# Autodesk Inventor assembly: robot arm
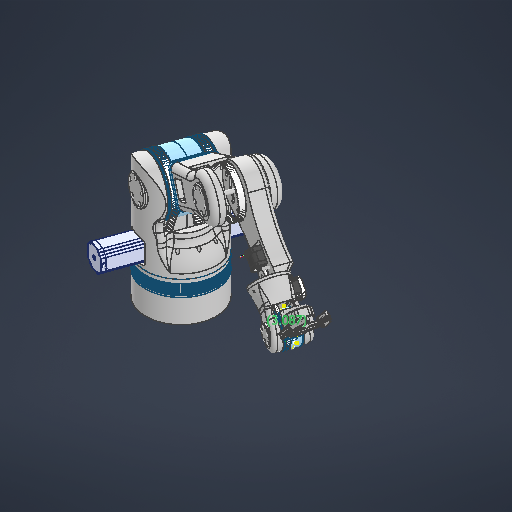
[picture p0: Inventor's stored thumbnail of the model, 512x512]
Saved by Autodesk Inventor 2026 (Build 300175000, 175)
## iProperties
Created: 2026-04-20
Part Number: robot arm
Document SubType Name: Assembly
Designer: oleg2
Author: oleg2
## Documents named in this file (35)
- E:\robot arm.iam
- E:\fasteners\m5 lock nut.ipt
- E:\fasteners\m5 washer.ipt
- E:\fasteners\m5 30mm screw.ipt
- E:\bottom piece.ipt
- E:\118t pulley part 2.ipt
- E:\bearing\outerbearingwheel.ipt
- E:\bearing\innerbearingwheel.ipt
- E:\middle piece.ipt
- E:\stepper motor.ipt
- E:\fasteners\m4 30mm screw.ipt
- E:\fasteners\m4 16mm flat head screw.ipt
- E:\fasteners\m5 hex nut.ipt
- E:\fasteners\m5 15mm screw.ipt
- E:\90t 1in pulley.ipt
- E:\rod.ipt
- E:\rodbearing.ipt
- E:\bearingplate.ipt
- E:\stepper motor 2.ipt
- E:\bearing 2.ipt
- E:\bearingplate 2.ipt
- E:\10mm rod.ipt
- E:\BELT LARGE.ipt
- E:\75t pulley (1).ipt
- E:\75t pulley right.ipt
- E:\final joint.ipt
- E:\3in 10mm rod.ipt
- E:\stepper 3.ipt
- E:\50t pulley.ipt
- E:\50t pulley right piece.ipt
- E:\bearing plate final.ipt
- E:\arm 2 fixed.ipt
- E:\epic claw.iam
- E:\107t belt.ipt
- E:\61t belt.ipt
## Components (115 placed, 34 different names)
1. m5 lock nut:1 — Mate:32, Mate:38
2. m5 washer:1 — Mate:20, Mate:24, Mate:39
3. m5 30mm screw:1 — Mate:10, Mate:12, Mate:26, Mate:33
4. bottom piece:1 — Mate:1, Mate:2, Mate:3, Mate:4, Mate:237
5. 118t pulley part 2:1 — Mate:1, Mate:6, Mate:18, Mate:19, Mate:20, Mate:21, Mate:22, Mate:23, Mate:24, Mate:25, Mate:40, Mate:41, Mate:42
6. outerbearingwheel:1 — Mate:2, Mate:3, Mate:4, Mate:5, Flush:1, Mate:61, Mate:62, Mate:63, Mate:64, Mate:65, Mate:66, Mate:67, Mate:68
7. innerbearingwheel:1 — Mate:5, Flush:1, Mate:6, Mate:7, Mate:8, Mate:9, Mate:10, Mate:15, Mate:16, Mate:17, Mate:25, Mate:27
8. m5 30mm screw:2 — Mate:7, Mate:11, Mate:29, Mate:32
9. m5 30mm screw:3 — Mate:8, Mate:14, Mate:30, Mate:31, Mate:35
10. m5 30mm screw:4 — Mate:9, Mate:13, Mate:28, Mate:34
11. m5 washer:2 — Mate:19, Mate:23, Mate:38
12. m5 washer:3 — Mate:18, Mate:31, Mate:36
13. m5 washer:4 — Mate:13, Mate:27, Mate:28
14. m5 washer:5 — Mate:12, Mate:16, Mate:26
15. m5 washer:6 — Mate:11, Mate:15, Mate:29
16. m5 washer:7 — Mate:14, Mate:17, Mate:30
17. m5 washer:8 — Mate:21, Mate:22, Mate:37
18. m5 lock nut:2 — Mate:33, Mate:39
19. m5 lock nut:3 — Mate:34, Mate:37
20. m5 lock nut:4 — Mate:35, Mate:36
21. middle piece:1 — Mate:40, Mate:41, Mate:42, Mate:43, Mate:44, Mate:45, Mate:46, Mate:47, Mate:48, Mate:49, Mate:50, Mate:51, Mate:52, Mate:53, Mate:54, Mate:55, Mate:56, Mate:57, Mate:58, Mate:59, Mate:60, Mate:69, Angle:1, Mate:70, Mate:71, Angle:2, Mate:72, Mate:73, Angle:3, Mate:74, Mate:75, Angle:4, Mate:76, Mate:77, Angle:5, Mate:78, Mate:79, Angle:6, Mate:80, Mate:81, Angle:7, Mate:82, Mate:83, Angle:8, Mate:84, Mate:89, Mate:104, Flush:3, Mate:130, Mate:131, Mate:203, Mate:205, Mate:206, Mate:238, Mate:239
22. stepper motor:1 — Mate:43, Mate:44, Mate:45, Mate:85, Mate:86, Mate:88, Mate:90, Mate:91, Mate:92, Mate:211
23. stepper motor:2 — Mate:46, Mate:47, Mate:48, Mate:93, Mate:94, Mate:95, Mate:96, Mate:97, Mate:98, Mate:99, Mate:100, Mate:208
24. m4 30mm screw:1 — Mate:49, Mate:50
25. m4 30mm screw:2 — Mate:51, Mate:52
26. m4 30mm screw:3 — Mate:53, Mate:54
27. m4 30mm screw:4 — Mate:55, Mate:56
28. m4 30mm screw:5 — Mate:57, Mate:58
29. m4 30mm screw:6 — Mate:59, Mate:60
30. m4 16mm flat head screw:1 — Mate:63, Mate:64
31. m4 16mm flat head screw:2 — Mate:61, Mate:62
32. m4 16mm flat head screw:3 — Mate:67, Mate:68
33. m4 16mm flat head screw:4 — Mate:65, Mate:66
34. m5 hex nut:1 — Mate:69, Angle:1, Mate:70
35. m5 hex nut:2 — Mate:71, Angle:2, Mate:72, Mate:87
36. m5 hex nut:3 — Mate:83, Angle:8, Mate:84
37. m5 hex nut:4 — Mate:81, Angle:7, Mate:82
38. m5 hex nut:5 — Mate:73, Angle:3, Mate:74
39. m5 hex nut:6 — Mate:75, Angle:4, Mate:76
40. m5 hex nut:7 — Mate:77, Angle:5, Mate:78
41. m5 hex nut:8 — Mate:79, Angle:6, Mate:80
42. m5 15mm screw:1 — Mate:91, Mate:92
43. m5 15mm screw:2 — Mate:87, Mate:88
44. m5 15mm screw:3 — Mate:93, Mate:94
45. m5 15mm screw:4 — Mate:89, Mate:90
46. m5 15mm screw:5 — Mate:97, Mate:98
47. m5 15mm screw:6 — Mate:95, Mate:96
48. m5 15mm screw:7 — Mate:99, Mate:100
49. m5 15mm screw:8 — Mate:85, Mate:86
50. 90t 1in pulley:1 — Mate:103, Mate:107, Mate:108, Mate:127, Mate:209, Mate:292
51. 90t 1in pulley:2 — Mate:103, Mate:104, Mate:107, Mate:119, Mate:120, Mate:121, Mate:122, Mate:123, Mate:124, Mate:125, Mate:126, Mate:127, Mate:212, Mate:291, Mate:293
52. rod:1 — Mate:108, Flush:3, Mate:109, Mate:111, Mate:113, Mate:118, Mate:203, Mate:207, Mate:210
53. rodbearing:1 — Mate:109, Mate:206
54. rodbearing:2 — Mate:111, Mate:205
55. bearingplate:1 — Mate:113, Mate:130, Mate:142, Mate:143, Mate:144, Mate:145, Mate:146, Mate:147, Mate:148, Mate:149, Mate:150, Mate:151
56. bearingplate:2 — Mate:118, Mate:131, Mate:132, Mate:133, Mate:134, Mate:135, Mate:136, Mate:137, Mate:138, Mate:139, Mate:140, Mate:141
57. m4 30mm screw:7 — Mate:119, Mate:120
58. m4 30mm screw:8 — Mate:121, Mate:122
59. m4 30mm screw:9 — Mate:123, Mate:124
60. m4 30mm screw:10 — Mate:125, Mate:126
61. m4 16mm flat head screw:5 — Mate:132, Mate:133, Mate:238
62. m4 16mm flat head screw:6 — Mate:134, Mate:135
63. m4 16mm flat head screw:7 — Mate:136, Mate:137
64. m4 16mm flat head screw:8 — Mate:150, Mate:151
65. m4 16mm flat head screw:9 — Mate:140, Mate:141
66. m4 16mm flat head screw:10 — Mate:138, Mate:139
67. m4 16mm flat head screw:12 — Mate:148, Mate:149
68. m4 16mm flat head screw:13 — Mate:142, Mate:143
69. m4 16mm flat head screw:14 — Mate:144, Mate:145
70. m4 16mm flat head screw:15 — Mate:146, Mate:147, Mate:239
71. stepper motor 2:1 — Mate:294, Mate:295, Mate:296, Mate:318
72. bearing 2:2 — Mate:175, Mate:290, Mate:299
73. bearingplate 2:1 — Mate:183, Mate:184, Mate:185, Mate:186, Mate:187, Mate:188, Mate:189, Mate:190, Mate:191, Mate:192, Mate:306
74. bearingplate 2:2 — Mate:175, Mate:193, Mate:194, Mate:195, Mate:196, Mate:197, Mate:198, Mate:199, Mate:200, Mate:201, Mate:202, Mate:204, Mate:300
75. 10mm rod:1 — Mate:290, Mate:302, Mate:311, Flush:5, Mate:317
76. m4 16mm flat head screw:16 — Mate:185, Mate:186
77. m4 16mm flat head screw:17 — Mate:187, Mate:188, Mate:304
78. m4 16mm flat head screw:18 — Mate:189, Mate:190, Mate:305
79. m4 16mm flat head screw:19 — Mate:195, Mate:196
80. m4 16mm flat head screw:20 — Mate:197, Mate:198
81. m4 16mm flat head screw:21 — Mate:201, Mate:202, Mate:204
82. m4 16mm flat head screw:22 — Mate:199, Mate:200
83. m4 16mm flat head screw:23 — Mate:193, Mate:194
84. m4 16mm flat head screw:24 — Mate:191, Mate:192
85. m4 16mm flat head screw:25 — Mate:183, Mate:184
86. BELT LARGE:1 — Mate:207, Mate:208, Mate:209
87. BELT LARGE:2 — Mate:210, Mate:211, Mate:212
88. 75t pulley (1):2 — Mate:236, Mate:250, Mate:308, Mate:309, Mate:320, Mate:322, Mate:323
89. stepper motor 2:2 — Mate:236, Mate:320, Mate:321
90. 75t pulley right:2 — Mate:307, Mate:308, Mate:309, Mate:310, Mate:313, Mate:321
91. final joint:1 — Mate:244, Mate:245, Mate:246, Flush:4, Mate:247, Mate:248, Mate:249, Mate:250, Mate:260, Mate:263, Mate:264, Mate:265, Mate:266, Mate:267, Mate:268, Mate:313
92. bearing 2:3 — Mate:241, Mate:246
93. 3in 10mm rod:1 — Mate:241, Mate:243, Mate:245, Flush:4, Mate:259, Mate:261
94. bearing 2:4 — Mate:243, Mate:244
95. stepper 3:1 — Mate:247, Mate:248, Mate:249, Mate:324
96. 50t pulley:1 — Mate:259, Mate:260, Mate:262, Mate:315, Mate:325, Mate:326
97. 50t pulley right piece:1 — Mate:261, Mate:262, Mate:314, Mate:316
98. bearing plate final:1 — Mate:263, Mate:264, Mate:265, Mate:269, Mate:270, Mate:271, Mate:272, Mate:273, Mate:274, Mate:275, Mate:276, Mate:277, Mate:278
99. bearing plate final:2 — Mate:266, Mate:267, Mate:268, Mate:279, Mate:280, Mate:281, Mate:282, Mate:283, Mate:284, Mate:285, Mate:286, Mate:287, Mate:288
100. m4 16mm flat head screw:26 — Mate:269, Mate:270
101. m4 16mm flat head screw:27 — Mate:279, Mate:280
102. m4 16mm flat head screw:28 — Mate:283, Mate:284
103. m4 16mm flat head screw:29 — Mate:287, Mate:288
104. m4 16mm flat head screw:30 — Mate:271, Mate:272
105. m4 16mm flat head screw:31 — Mate:285, Mate:286
106. m4 16mm flat head screw:32 — Mate:273, Mate:274
107. m4 16mm flat head screw:33 — Mate:275, Mate:276
108. m4 16mm flat head screw:34 — Mate:277, Mate:278
109. m4 16mm flat head screw:35 — Mate:281, Mate:282
110. arm 2 fixed:1 — Mate:291, Mate:292, Mate:293, Mate:294, Mate:295, Mate:296, Mate:299, Mate:300, Mate:301, Mate:304, Mate:305, Mate:306, Mate:307, Mate:310, Mate:311, Mate:319
111. bearing 2:5 — Mate:301, Mate:302, Flush:5
112. epic claw:1 [sub-assembly] — Mate:314, Mate:315, Mate:316
113. 107t belt:1 — Mate:317, Mate:318, Mate:319
114. m4 30mm screw:11 — Mate:322, Mate:323
115. 61t belt:1 — Mate:324, Mate:325, Mate:326
## Relationships (259: Mate 246, Angle 8, Flush 5)
- Mate:1: bottom piece:1 ↔ 118t pulley part 2:1
- Mate:2: bottom piece:1 ↔ outerbearingwheel:1
- Mate:3: bottom piece:1 ↔ outerbearingwheel:1
- Mate:4: bottom piece:1 ↔ outerbearingwheel:1
- Mate:5: outerbearingwheel:1 ↔ innerbearingwheel:1
- Flush:1: outerbearingwheel:1 ↔ innerbearingwheel:1
- Mate:6: 118t pulley part 2:1 ↔ innerbearingwheel:1
- Mate:7: innerbearingwheel:1 ↔ m5 30mm screw:2
- Mate:8: innerbearingwheel:1 ↔ m5 30mm screw:3
- Mate:9: innerbearingwheel:1 ↔ m5 30mm screw:4
- Mate:10: m5 30mm screw:1 ↔ innerbearingwheel:1
- Mate:11: m5 30mm screw:2 ↔ m5 washer:6
- Mate:12: m5 30mm screw:1 ↔ m5 washer:5
- Mate:13: m5 30mm screw:4 ↔ m5 washer:4
- Mate:14: m5 30mm screw:3 ↔ m5 washer:7
- Mate:15: innerbearingwheel:1 ↔ m5 washer:6
- Mate:16: innerbearingwheel:1 ↔ m5 washer:5
- Mate:17: innerbearingwheel:1 ↔ m5 washer:7
- Mate:18: 118t pulley part 2:1 ↔ m5 washer:3
- Mate:19: 118t pulley part 2:1 ↔ m5 washer:2
- Mate:20: m5 washer:1 ↔ 118t pulley part 2:1
- Mate:21: 118t pulley part 2:1 ↔ m5 washer:8
- Mate:22: 118t pulley part 2:1 ↔ m5 washer:8
- Mate:23: 118t pulley part 2:1 ↔ m5 washer:2
- Mate:24: m5 washer:1 ↔ 118t pulley part 2:1
- Mate:25: 118t pulley part 2:1 ↔ innerbearingwheel:1
- Mate:26: m5 30mm screw:1 ↔ m5 washer:5
- Mate:27: innerbearingwheel:1 ↔ m5 washer:4
- Mate:28: m5 30mm screw:4 ↔ m5 washer:4
- Mate:29: m5 30mm screw:2 ↔ m5 washer:6
- Mate:30: m5 30mm screw:3 ↔ m5 washer:7
- Mate:31: m5 30mm screw:3 ↔ m5 washer:3
- Mate:32: m5 lock nut:1 ↔ m5 30mm screw:2
- Mate:33: m5 30mm screw:1 ↔ m5 lock nut:2
- Mate:34: m5 30mm screw:4 ↔ m5 lock nut:3
- Mate:35: m5 30mm screw:3 ↔ m5 lock nut:4
- Mate:36: m5 washer:3 ↔ m5 lock nut:4
- Mate:37: m5 washer:8 ↔ m5 lock nut:3
- Mate:38: m5 lock nut:1 ↔ m5 washer:2
- Mate:39: m5 washer:1 ↔ m5 lock nut:2
- Mate:40: 118t pulley part 2:1 ↔ middle piece:1
- Mate:41: 118t pulley part 2:1 ↔ middle piece:1
- Mate:42: 118t pulley part 2:1 ↔ middle piece:1
- Mate:43: middle piece:1 ↔ stepper motor:1
- Mate:44: middle piece:1 ↔ stepper motor:1
- Mate:45: middle piece:1 ↔ stepper motor:1
- Mate:46: middle piece:1 ↔ stepper motor:2
- Mate:47: middle piece:1 ↔ stepper motor:2
- Mate:48: middle piece:1 ↔ stepper motor:2
- Mate:49: middle piece:1 ↔ m4 30mm screw:1
- Mate:50: middle piece:1 ↔ m4 30mm screw:1
- Mate:51: middle piece:1 ↔ m4 30mm screw:2
- Mate:52: middle piece:1 ↔ m4 30mm screw:2
- Mate:53: middle piece:1 ↔ m4 30mm screw:3
- Mate:54: middle piece:1 ↔ m4 30mm screw:3
- Mate:55: middle piece:1 ↔ m4 30mm screw:4
- Mate:56: middle piece:1 ↔ m4 30mm screw:4
- Mate:57: middle piece:1 ↔ m4 30mm screw:5
- Mate:58: middle piece:1 ↔ m4 30mm screw:5
- Mate:59: middle piece:1 ↔ m4 30mm screw:6
- Mate:60: middle piece:1 ↔ m4 30mm screw:6
- Mate:61: outerbearingwheel:1 ↔ m4 16mm flat head screw:2
- Mate:62: outerbearingwheel:1 ↔ m4 16mm flat head screw:2
- Mate:63: outerbearingwheel:1 ↔ m4 16mm flat head screw:1
- Mate:64: outerbearingwheel:1 ↔ m4 16mm flat head screw:1
- Mate:65: outerbearingwheel:1 ↔ m4 16mm flat head screw:4
- Mate:66: outerbearingwheel:1 ↔ m4 16mm flat head screw:4
- Mate:67: outerbearingwheel:1 ↔ m4 16mm flat head screw:3
- Mate:68: outerbearingwheel:1 ↔ m4 16mm flat head screw:3
- Mate:69: middle piece:1 ↔ m5 hex nut:1
- Angle:1 (0 deg): middle piece:1 ↔ m5 hex nut:1
- Mate:70: middle piece:1 ↔ m5 hex nut:1
- Mate:71: middle piece:1 ↔ m5 hex nut:2
- Angle:2 (0 deg): middle piece:1 ↔ m5 hex nut:2
- Mate:72: middle piece:1 ↔ m5 hex nut:2
- Mate:73: middle piece:1 ↔ m5 hex nut:5
- Angle:3 (0 deg): middle piece:1 ↔ m5 hex nut:5
- Mate:74: middle piece:1 ↔ m5 hex nut:5
- Mate:75: middle piece:1 ↔ m5 hex nut:6
- Angle:4 (0 deg): middle piece:1 ↔ m5 hex nut:6
- Mate:76: middle piece:1 ↔ m5 hex nut:6
- Mate:77: middle piece:1 ↔ m5 hex nut:7
- Angle:5 (0 deg): middle piece:1 ↔ m5 hex nut:7
- Mate:78: middle piece:1 ↔ m5 hex nut:7
- Mate:79: middle piece:1 ↔ m5 hex nut:8
- Angle:6 (0 deg): middle piece:1 ↔ m5 hex nut:8
- Mate:80: middle piece:1 ↔ m5 hex nut:8
- Mate:81: middle piece:1 ↔ m5 hex nut:4
- Angle:7 (0 deg): middle piece:1 ↔ m5 hex nut:4
- Mate:82: middle piece:1 ↔ m5 hex nut:4
- Mate:83: middle piece:1 ↔ m5 hex nut:3
- Angle:8 (0 deg): middle piece:1 ↔ m5 hex nut:3
- Mate:84: middle piece:1 ↔ m5 hex nut:3
- Mate:85: stepper motor:1 ↔ m5 15mm screw:8
- Mate:86: stepper motor:1 ↔ m5 15mm screw:8
- Mate:87: m5 hex nut:2 ↔ m5 15mm screw:2
- Mate:88: stepper motor:1 ↔ m5 15mm screw:2
- Mate:89: middle piece:1 ↔ m5 15mm screw:4
- Mate:90: stepper motor:1 ↔ m5 15mm screw:4
- Mate:91: stepper motor:1 ↔ m5 15mm screw:1
- Mate:92: stepper motor:1 ↔ m5 15mm screw:1
- Mate:93: stepper motor:2 ↔ m5 15mm screw:3
- Mate:94: stepper motor:2 ↔ m5 15mm screw:3
- Mate:95: stepper motor:2 ↔ m5 15mm screw:6
- Mate:96: stepper motor:2 ↔ m5 15mm screw:6
- Mate:97: stepper motor:2 ↔ m5 15mm screw:5
- Mate:98: stepper motor:2 ↔ m5 15mm screw:5
- Mate:99: stepper motor:2 ↔ m5 15mm screw:7
- Mate:100: stepper motor:2 ↔ m5 15mm screw:7
- Flush:2 (233.3625 mm)
- Mate:103: 90t 1in pulley:1 ↔ 90t 1in pulley:2
- Mate:104 (1.5621 mm): middle piece:1 ↔ 90t 1in pulley:2
- Mate:107: 90t 1in pulley:1 ↔ 90t 1in pulley:2
- Mate:108: 90t 1in pulley:1 ↔ rod:1
- Flush:3: middle piece:1 ↔ rod:1
- Mate:109: rod:1 ↔ rodbearing:1
- Mate:111: rod:1 ↔ rodbearing:2
- Mate:113: rod:1 ↔ bearingplate:1
- Mate:118: rod:1 ↔ bearingplate:2
- Mate:119: 90t 1in pulley:2 ↔ m4 30mm screw:7
- Mate:120: 90t 1in pulley:2 ↔ m4 30mm screw:7
- Mate:121: 90t 1in pulley:2 ↔ m4 30mm screw:8
- Mate:122: 90t 1in pulley:2 ↔ m4 30mm screw:8
- Mate:123: 90t 1in pulley:2 ↔ m4 30mm screw:9
- Mate:124: 90t 1in pulley:2 ↔ m4 30mm screw:9
- Mate:125: 90t 1in pulley:2 ↔ m4 30mm screw:10
- Mate:126: 90t 1in pulley:2 ↔ m4 30mm screw:10
- Mate:127: 90t 1in pulley:1 ↔ 90t 1in pulley:2
- Mate:130: middle piece:1 ↔ bearingplate:1
- Mate:131: middle piece:1 ↔ bearingplate:2
- Mate:132: bearingplate:2 ↔ m4 16mm flat head screw:5
- Mate:133: bearingplate:2 ↔ m4 16mm flat head screw:5
- Mate:134: bearingplate:2 ↔ m4 16mm flat head screw:6
- Mate:135: bearingplate:2 ↔ m4 16mm flat head screw:6
- Mate:136: bearingplate:2 ↔ m4 16mm flat head screw:7
- Mate:137: bearingplate:2 ↔ m4 16mm flat head screw:7
- Mate:138: bearingplate:2 ↔ m4 16mm flat head screw:10
- Mate:139: bearingplate:2 ↔ m4 16mm flat head screw:10
- Mate:140: bearingplate:2 ↔ m4 16mm flat head screw:9
- Mate:141: bearingplate:2 ↔ m4 16mm flat head screw:9
- Mate:142: bearingplate:1 ↔ m4 16mm flat head screw:13
- Mate:143: bearingplate:1 ↔ m4 16mm flat head screw:13
- Mate:144: bearingplate:1 ↔ m4 16mm flat head screw:14
- Mate:145: bearingplate:1 ↔ m4 16mm flat head screw:14
- Mate:146: bearingplate:1 ↔ m4 16mm flat head screw:15
- Mate:147: bearingplate:1 ↔ m4 16mm flat head screw:15
- Mate:148: bearingplate:1 ↔ m4 16mm flat head screw:12
- Mate:149: bearingplate:1 ↔ m4 16mm flat head screw:12
- Mate:150: bearingplate:1 ↔ m4 16mm flat head screw:8
- Mate:151: bearingplate:1 ↔ m4 16mm flat head screw:8
- Mate:175: bearing 2:2 ↔ bearingplate 2:2
- Mate:183: bearingplate 2:1 ↔ m4 16mm flat head screw:25
- Mate:184: bearingplate 2:1 ↔ m4 16mm flat head screw:25
- Mate:185: bearingplate 2:1 ↔ m4 16mm flat head screw:16
- Mate:186: bearingplate 2:1 ↔ m4 16mm flat head screw:16
- Mate:187: bearingplate 2:1 ↔ m4 16mm flat head screw:17
- Mate:188: bearingplate 2:1 ↔ m4 16mm flat head screw:17
- Mate:189: bearingplate 2:1 ↔ m4 16mm flat head screw:18
- Mate:190: bearingplate 2:1 ↔ m4 16mm flat head screw:18
- Mate:191: bearingplate 2:1 ↔ m4 16mm flat head screw:24
- Mate:192: bearingplate 2:1 ↔ m4 16mm flat head screw:24
- Mate:193: bearingplate 2:2 ↔ m4 16mm flat head screw:23
- Mate:194: bearingplate 2:2 ↔ m4 16mm flat head screw:23
- Mate:195: bearingplate 2:2 ↔ m4 16mm flat head screw:19
- Mate:196: bearingplate 2:2 ↔ m4 16mm flat head screw:19
- Mate:197: bearingplate 2:2 ↔ m4 16mm flat head screw:20
- Mate:198: bearingplate 2:2 ↔ m4 16mm flat head screw:20
- Mate:199: bearingplate 2:2 ↔ m4 16mm flat head screw:22
- Mate:200: bearingplate 2:2 ↔ m4 16mm flat head screw:22
- Mate:201: bearingplate 2:2 ↔ m4 16mm flat head screw:21
- Mate:202: bearingplate 2:2 ↔ m4 16mm flat head screw:21
- Mate:203: middle piece:1 ↔ rod:1
- Mate:204: bearingplate 2:2 ↔ m4 16mm flat head screw:21
- Mate:205: middle piece:1 ↔ rodbearing:2
- Mate:206: middle piece:1 ↔ rodbearing:1
- Mate:207: rod:1 ↔ BELT LARGE:1
- Mate:208: stepper motor:2 ↔ BELT LARGE:1
- Mate:209 (3.81 mm): 90t 1in pulley:1 ↔ BELT LARGE:1
- Mate:210: rod:1 ↔ BELT LARGE:2
- Mate:211: stepper motor:1 ↔ BELT LARGE:2
- Mate:212 (3.81 mm): 90t 1in pulley:2 ↔ BELT LARGE:2
- Mate:236: 75t pulley (1):2 ↔ stepper motor 2:2
- Mate:237: bottom piece:1
- Mate:238: middle piece:1 ↔ m4 16mm flat head screw:5
- Mate:239: middle piece:1 ↔ m4 16mm flat head screw:15
- Mate:241: bearing 2:3 ↔ 3in 10mm rod:1
- Mate:243: 3in 10mm rod:1 ↔ bearing 2:4
- Mate:244: final joint:1 ↔ bearing 2:4
- Mate:245: final joint:1 ↔ 3in 10mm rod:1
- Mate:246: final joint:1 ↔ bearing 2:3
- Flush:4: final joint:1 ↔ 3in 10mm rod:1
- Mate:247: final joint:1 ↔ stepper 3:1
- Mate:248: final joint:1 ↔ stepper 3:1
- Mate:249: final joint:1 ↔ stepper 3:1
- Mate:250: 75t pulley (1):2 ↔ final joint:1
- Mate:259: 3in 10mm rod:1 ↔ 50t pulley:1
- Mate:260 (1.905 mm): final joint:1 ↔ 50t pulley:1
- Mate:261: 3in 10mm rod:1 ↔ 50t pulley right piece:1
- Mate:262: 50t pulley:1 ↔ 50t pulley right piece:1
- Mate:263: final joint:1 ↔ bearing plate final:1
- Mate:264: final joint:1 ↔ bearing plate final:1
- Mate:265: final joint:1 ↔ bearing plate final:1
- Mate:266: final joint:1 ↔ bearing plate final:2
- Mate:267: final joint:1 ↔ bearing plate final:2
- Mate:268: final joint:1 ↔ bearing plate final:2
- Mate:269: bearing plate final:1 ↔ m4 16mm flat head screw:26
- Mate:270: bearing plate final:1 ↔ m4 16mm flat head screw:26
- Mate:271: bearing plate final:1 ↔ m4 16mm flat head screw:30
- Mate:272: bearing plate final:1 ↔ m4 16mm flat head screw:30
- Mate:273: bearing plate final:1 ↔ m4 16mm flat head screw:32
- Mate:274: bearing plate final:1 ↔ m4 16mm flat head screw:32
- Mate:275: bearing plate final:1 ↔ m4 16mm flat head screw:33
- Mate:276: bearing plate final:1 ↔ m4 16mm flat head screw:33
- Mate:277: bearing plate final:1 ↔ m4 16mm flat head screw:34
- Mate:278: bearing plate final:1 ↔ m4 16mm flat head screw:34
- Mate:279: bearing plate final:2 ↔ m4 16mm flat head screw:27
- Mate:280: bearing plate final:2 ↔ m4 16mm flat head screw:27
- Mate:281: bearing plate final:2 ↔ m4 16mm flat head screw:35
- Mate:282: bearing plate final:2 ↔ m4 16mm flat head screw:35
- Mate:283: bearing plate final:2 ↔ m4 16mm flat head screw:28
- Mate:284: bearing plate final:2 ↔ m4 16mm flat head screw:28
- Mate:285: bearing plate final:2 ↔ m4 16mm flat head screw:31
- Mate:286: bearing plate final:2 ↔ m4 16mm flat head screw:31
- Mate:287: bearing plate final:2 ↔ m4 16mm flat head screw:29
- Mate:288: bearing plate final:2 ↔ m4 16mm flat head screw:29
- Mate:290: bearing 2:2 ↔ 10mm rod:1
- Mate:291: 90t 1in pulley:2 ↔ arm 2 fixed:1
- Mate:292: 90t 1in pulley:1 ↔ arm 2 fixed:1
- Mate:293: 90t 1in pulley:2 ↔ arm 2 fixed:1
- Mate:294: stepper motor 2:1 ↔ arm 2 fixed:1
- Mate:295: stepper motor 2:1 ↔ arm 2 fixed:1
- Mate:296: stepper motor 2:1 ↔ arm 2 fixed:1
- Mate:299: bearing 2:2 ↔ arm 2 fixed:1
- Mate:300: bearingplate 2:2 ↔ arm 2 fixed:1
- Mate:301: arm 2 fixed:1 ↔ bearing 2:5
- Mate:302: 10mm rod:1 ↔ bearing 2:5
- Mate:304: m4 16mm flat head screw:17 ↔ arm 2 fixed:1
- Mate:305: m4 16mm flat head screw:18 ↔ arm 2 fixed:1
- Mate:306: bearingplate 2:1 ↔ arm 2 fixed:1
- Mate:307 (1.27 mm): 75t pulley right:2 ↔ arm 2 fixed:1
- Mate:308: 75t pulley (1):2 ↔ 75t pulley right:2
- Mate:309: 75t pulley (1):2 ↔ 75t pulley right:2
- Mate:310: 75t pulley right:2 ↔ arm 2 fixed:1
- Mate:311: 10mm rod:1 ↔ arm 2 fixed:1
- Flush:5: 10mm rod:1 ↔ bearing 2:5
- Mate:313: 75t pulley right:2 ↔ final joint:1
- Mate:314: 50t pulley right piece:1 ↔ epic claw:1
- Mate:315: 50t pulley:1 ↔ epic claw:1
- Mate:316: 50t pulley right piece:1 ↔ epic claw:1
- Mate:317: 10mm rod:1 ↔ 107t belt:1
- Mate:318: stepper motor 2:1 ↔ 107t belt:1
- Mate:319 (3.81 mm): arm 2 fixed:1 ↔ 107t belt:1
- Mate:320: 75t pulley (1):2 ↔ stepper motor 2:2
- Mate:321: stepper motor 2:2 ↔ 75t pulley right:2
- Mate:322: 75t pulley (1):2 ↔ m4 30mm screw:11
- Mate:323: 75t pulley (1):2 ↔ m4 30mm screw:11
- Mate:324: stepper 3:1 ↔ 61t belt:1
- Mate:325: 50t pulley:1 ↔ 61t belt:1
- Mate:326 (1.27 mm): 50t pulley:1 ↔ 61t belt:1
